# Autodesk Inventor assembly: Turret Assembly
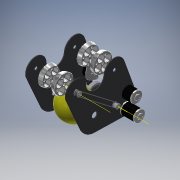
[picture p0: Inventor's stored thumbnail of the model, 180x180]
Saved by Autodesk Inventor 2019.4 (Build 234330000, 330)
## iProperties
Created: 2020-01-16
Part Number: Turret Assembly
Document SubType Name: Assembly
Designer: admin
Mass: 7034.5 g
Surface Area: 8289.28 cm^2
Volume: 5614.99 cm^3
Density: 1.25281 g/cm^3
Author: admin
## Documents named in this file (10)
- C:\Users\admin\Desktop\FRC 2020 Engineering\GitHub\7738-2020\Robot V2\Turret\Turret Assembly.iam
- C:\Users\admin\Desktop\FRC 2020 Engineering\GitHub\7738-2020\Robot V2\Turret\Flywheel Half.ipt
- C:\Users\admin\Desktop\FRC 2020 Engineering\GitHub\7738-2020\Robot V2\Turret\Colson_Performa_4_x_0_875_1_2_Hex_bore_217-4049.ipt
- C:\Users\admin\Desktop\FRC 2020 Engineering\GitHub\7738-2020\Robot V2\Turret\Shooter Side Plate.ipt
- C:\Users\admin\Desktop\FRC 2020 Engineering\GitHub\7738-2020\Robot V2\Turret\Mini_CIM_Motor_217-3371.ipt
- C:\Users\admin\Desktop\FRC 2020 Engineering\GitHub\7738-2020\Power Cell.ipt
- C:\Users\admin\Desktop\FRC 2020 Engineering\GitHub\7738-2020\Robot V2\Turret\Motor Mount.ipt
- C:\Users\admin\Desktop\FRC 2020 Engineering\GitHub\7738-2020\Robot V2\Turret\Turret Assembly\Design Accelerator\Synchronous Belts Transmission2.iam
- C:\Users\admin\Desktop\FRC 2020 Engineering\GitHub\7738-2020\Robot V2\Turret\Turret Assembly\Design Accelerator\Synchronous Belts Transmission3.iam
- C:\Users\admin\Desktop\FRC 2020 Engineering\GitHub\7738-2020\Robot V2\Turret\Turret Assembly\Design Accelerator\Synchronous Belts Transmission4.iam
## Components (17 placed, 7 different names)
1. Shooter Side Plate:1 — Mate:34, Mate:38, Mate:39, Mate:43, Mate:45, Mate:49, Mate:51, Mate:53, Mate:58, Mate:60, Angle:1
2. Colson_Performa_4_x_0_875_1_2_Hex_bore_217-4049:3 — Mate:45, Mate:46
3. Flywheel Half:11 — Mate:35, Mate:36, Mate:37, Mate:38, Mate:47
4. Flywheel Half:12 — Mate:35, Mate:36
5. Flywheel Half:13 — Mate:42, Mate:43, Mate:48
6. Flywheel Half:14
7. Power Cell:1 — Mate:44
8. Shooter Side Plate:2 — Mate:47, Mate:48, Mate:49, Mate:55, Mate:57, Mate:62, Mate:65, Angle:2
9. Mini_CIM_Motor_217-3371:6 — Mate:51, Mate:53
10. Mini_CIM_Motor_217-3371:8 — Mate:55, Mate:57
11. Mini_CIM_Motor_217-3371:9 — Mate:63, Mate:64, Mate:65
12. Mini_CIM_Motor_217-3371:10 — Mate:59, Mate:60, Mate:61
13. Motor Mount:1 — Mate:58, Mate:59, Mate:61, Angle:1
14. Motor Mount:2 — Mate:62, Mate:63, Mate:64, Angle:2
15. Synchronous Belts Transmission:1 [sub-assembly]
16. Synchronous Belts Transmission:2 [sub-assembly]
17. Synchronous Belts Transmission:3 [sub-assembly]
## Relationships (30: Mate 28, Angle 2)
- Mate:34 (114.3 mm): Shooter Side Plate:1
- Mate:35: Flywheel Half:11 ↔ Flywheel Half:12
- Mate:36 (50 mm): Flywheel Half:11 ↔ Flywheel Half:12
- Mate:37 (25 mm): Flywheel Half:11
- Mate:38: Shooter Side Plate:1 ↔ Flywheel Half:11
- Mate:39: Shooter Side Plate:1
- [Mate]: Flywheel Half:13 ↔ Flywheel Half:14
- [Mate] (50 mm): Flywheel Half:13 ↔ Flywheel Half:14
- Mate:42 (25 mm): Flywheel Half:13
- Mate:43: Shooter Side Plate:1 ↔ Flywheel Half:13
- Mate:44: Power Cell:1
- Mate:45: Shooter Side Plate:1 ↔ Colson_Performa_4_x_0_875_1_2_Hex_bore_217-4049:3
- Mate:46: Colson_Performa_4_x_0_875_1_2_Hex_bore_217-4049:3
- Mate:47: Flywheel Half:11 ↔ Shooter Side Plate:2
- Mate:48: Flywheel Half:13 ↔ Shooter Side Plate:2
- Mate:49 (228.6 mm): Shooter Side Plate:1 ↔ Shooter Side Plate:2
- Mate:51: Shooter Side Plate:1 ↔ Mini_CIM_Motor_217-3371:6
- Mate:53: Shooter Side Plate:1 ↔ Mini_CIM_Motor_217-3371:6
- Mate:55: Shooter Side Plate:2 ↔ Mini_CIM_Motor_217-3371:8
- Mate:57: Shooter Side Plate:2 ↔ Mini_CIM_Motor_217-3371:8
- Mate:58 (25 mm): Shooter Side Plate:1 ↔ Motor Mount:1
- Mate:59: Mini_CIM_Motor_217-3371:10 ↔ Motor Mount:1
- Mate:60: Shooter Side Plate:1 ↔ Mini_CIM_Motor_217-3371:10
- Mate:61: Mini_CIM_Motor_217-3371:10 ↔ Motor Mount:1
- Angle:1 (0 deg): Shooter Side Plate:1 ↔ Motor Mount:1
- Mate:62 (25 mm): Shooter Side Plate:2 ↔ Motor Mount:2
- Mate:63: Mini_CIM_Motor_217-3371:9 ↔ Motor Mount:2
- Mate:64: Mini_CIM_Motor_217-3371:9 ↔ Motor Mount:2
- Mate:65: Shooter Side Plate:2 ↔ Mini_CIM_Motor_217-3371:9
- Angle:2 (0 deg): Shooter Side Plate:2 ↔ Motor Mount:2
## Named parameters: d73_d68 = 0 mm, d74_d69 = 50 mm
